# Autodesk Inventor assembly: SHOE_ASM
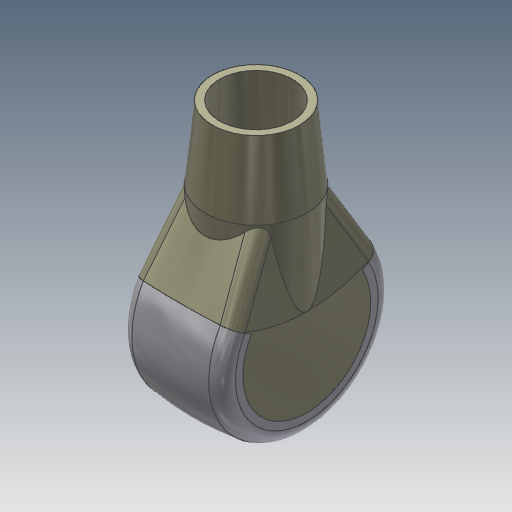
[picture p0: Inventor's stored thumbnail of the model, 512x512]
Saved by Autodesk Inventor 2019.4 (Build 234330000, 330)
## iProperties
Created: 2020-02-11
Part Number: SHOE_ASM
Material: 一般
Document SubType Name: Assembly
Designer: y6tada
Mass: 6.94447 g
Surface Area: 43.5356 cm^2
Volume: 6.21509 cm^3
Density: 1.11736 g/cm^3
Author: y6tada
## Documents named in this file (3)
- C:\Workspace\HaptHexa\Hardware\Inventor\Tibia\SHOE_ASM.iam
- C:\Workspace\HaptHexa\Hardware\Inventor\Tibia\GRIP_BASE_V2.ipt
- C:\Workspace\HaptHexa\Hardware\Inventor\GRIP_RUBBER.ipt
## Components (2 placed, 2 different names)
1. GRIP_BASE_V2:1
2. GRIP_RUBBER:1 — フラッシュ:1
## Relationships (1: Flush 1)
- フラッシュ:1 [Flush]: GRIP_RUBBER:1
